# Autodesk Inventor assembly: Z-head-assembly-IKO-T1
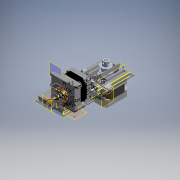
[picture p0: Inventor's stored thumbnail of the model, 180x180]
Saved by Autodesk Inventor 2016 (Build 200138000, 138)
## iProperties
Created: 2015-05-08
Part Number: Z-head-assembly-IKO-T1
Document SubType Name: Assembly
Designer: ax
Mass: 168.819 g
Surface Area: 717.643 cm^2
Volume: 138.854 cm^3
Density: 1.2158 g/cm^3
Author: ax
## Documents named in this file (24)
- C:\Users\as\Documents\Inventor\mintplacer-export\Z-head-assembly-IKO-T1.iam
- C:\Users\as\Documents\Inventor\mintplacer-export\Z-head-baseplate-IKO.ipt
- C:\Users\as\Documents\Inventor\mintplacer-export\BSPG15_60__40_.iam
- C:\Users\as\Documents\Inventor\mintplacer-export\C-head-base.ipt
- C:\Users\as\Documents\Inventor\mintplacer-export\C-head-side.ipt
- C:\Users\as\Documents\Inventor\mintplacer-export\GT2_20tooth.ipt
- C:\Users\as\Documents\Inventor\mintplacer-export\GT2-belt-2MR-200-06.ipt
- C:\Users\as\Documents\Inventor\mintplacer-export\HTD-5M-belt-clamp.ipt
- C:\Users\as\Documents\Inventor\mintplacer-export\GT2 belt clamp.ipt
- C:\Users\as\Documents\Inventor\mintplacer-export\NEMA14-Nanotec-ST3518S0804.ipt
- C:\Users\as\Documents\Inventor\mintplacer-export\nozzle-assembly.iam
- C:\Users\as\Documents\Inventor\mintplacer-export\Nanotec-ST4118S1404.iam
- C:\Users\as\Documents\Inventor\mintplacer-export\c-head-flange.ipt
- C:\Users\as\Documents\Inventor\mintplacer-export\Z-head-assembly-IKO-T1\Design Accelerator\Bolted Connection3.iam
- C:\Users\as\Documents\Inventor\mintplacer-export\Z-head-assembly-IKO-T1\Design Accelerator\Bolted Connection4.iam
- C:\Users\as\Documents\Inventor\mintplacer-export\Z-head-assembly-IKO-T1\Design Accelerator\Bolted Connection5.iam
- C:\Users\as\Documents\Inventor\mintplacer-export\Z-head-assembly-IKO-T1\Design Accelerator\Bolted Connection6.iam
- C:\Users\as\Documents\Inventor\mintplacer-export\Z-head-assembly-IKO-T1\Design Accelerator\Bolted Connection7.iam
- C:\Users\as\Documents\Inventor\mintplacer-export\small-tact-switch.ipt
- C:\Users\as\Documents\Inventor\mintplacer-export\Z-head-assembly-IKO-T1\Design Accelerator\Bolted Connection8.iam
- C:\Users\as\Documents\Inventor\mintplacer-export\Z-head-assembly-IKO-T1\Design Accelerator\Bolted Connection9.iam
- C:\Users\as\Documents\Inventor\mintplacer-export\Z-head-assembly-IKO-T1\Design Accelerator\Bolted Connection10.iam
- C:\Users\as\Documents\Inventor\mintplacer-export\Z-head-assembly-IKO-T1\Design Accelerator\Bolted Connection11.iam
- C:\Users\as\Documents\Inventor\Content Center Files\R2016\en-US\ISO 4762(1)\DIN EN ISO 4762 - M3 x 12.ipt
## Components (35 placed, 15 different names)
1. Z-head-baseplate-IKO:1 — Mate:1, Flush:1, Flush:2, Flush:7, Mate:5, Flush:9, Flush:10, Mate:10, Mate:37, Mate:38, Mate:39, Mate:40, Mate:41, Flush:21, Mate:70, Mate:71, Mate:74, Mate:76
2. HTD-5M-belt-clamp:1 — Flush:9, Flush:10
3. Nanotec-ST4118S1404:2 [sub-assembly] — Mate:5, Mate:10, Cylindrical:1, Flush:21, Mate:72, Mate:73, Mate:75
4. GT2_20tooth:1 — Mate:4, Cylindrical:1
5. BSPG15_60__40_:1 [sub-assembly] — Mate:1, Flush:1, Flush:2, Flush:3, Mate:11, Flush:19, Flush:20, Mate:43, Mate:69
6. c-head-flange:1 — Flush:14, Flush:15, Mate:11, Mate:12, Flush:17, Flush:19, Mate:32, Mate:33, Mate:34, Flush:20, Mate:42, Mate:47, Mate:52, Mate:53, Mate:68
7. C-head-base:1 — Flush:3, Flush:13, Mate:8, Mate:9, Flush:14, Flush:15, Flush:18, Mate:17, Mate:45
8. C-head-side:1 — Mate:7, Flush:11, Flush:13, Mate:12, Flush:17, Flush:18, Mate:17, Mate:44, Mate:46
9. NEMA14-Nanotec-ST3518S0804:1 — Mate:8, Mate:9
10. nozzle-assembly:1 [sub-assembly]
11. GT2 belt clamp:1 — Mate:7, Flush:11, Mate:48, Mate:49
12. Bolted Connection:3 [sub-assembly] — Mate:44, Mate:45
13. Bolted Connection:4 [sub-assembly] — Mate:46, Mate:47
14. Bolted Connection:5 [sub-assembly] — Mate:48, Mate:49
15. Bolted Connection:6 [sub-assembly] — Mate:68, Mate:69
16. Bolted Connection:7 [sub-assembly] — Mate:42, Mate:43
17. small-tact-switch:1 — Mate:32, Mate:33, Mate:34, Mate:62, Mate:63
18. Bolted Connection:8 [sub-assembly] — Mate:52, Mate:53
19. small-tact-switch:2 — Mate:37, Mate:38, Mate:66, Mate:67
20. small-tact-switch:3 — Mate:39, Mate:40, Mate:41, Mate:64, Mate:65
21. Bolted Connection:9 [sub-assembly] — Mate:62, Mate:63
22. Bolted Connection:10 [sub-assembly] — Mate:64, Mate:65
23. Bolted Connection:12 [sub-assembly] — Mate:66, Mate:67
24. DIN EN ISO 4762 M3 x 12:1 — Mate:70
25. DIN EN ISO 4762 M3 x 12:2 — Mate:71, Mate:72
26. DIN EN ISO 4762 M3 x 12:3 — Mate:74, Mate:75
27. DIN EN ISO 4762 M3 x 12:4 — Mate:73, Mate:76
28. GT2-belt-2MR-200-06:1 — Mate:4, Mate:6
29. GT2-belt-2MR-200-06:2
30. GT2-belt-2MR-200-06:3
31. GT2-belt-2MR-200-06:4
32. GT2-belt-2MR-200-06:5
33. GT2-belt-2MR-200-06:6
34. GT2-belt-2MR-200-06:7
35. GT2-belt-2MR-200-06:8
## Component patterns: (8 elements, first: GT2-belt-2MR-200-06:1)
## Relationships (61: Mate 44, Flush 16, CylindricalJoint 1)
- Mate:1: Z-head-baseplate-IKO:1 ↔ BSPG15_60__40_:1
- Flush:1: Z-head-baseplate-IKO:1 ↔ BSPG15_60__40_:1
- Flush:2: Z-head-baseplate-IKO:1 ↔ BSPG15_60__40_:1
- Flush:3: BSPG15_60__40_:1 ↔ C-head-base:1
- Mate:4 (1.4 mm): GT2_20tooth:1 ↔ GT2-belt-2MR-200-06:1
- Flush:7 (-6.3662 mm): Z-head-baseplate-IKO:1
- Mate:5 (-21 mm): Z-head-baseplate-IKO:1 ↔ Nanotec-ST4118S1404:2
- Flush:8 (-1.15 mm)
- Mate:6: GT2-belt-2MR-200-06:1
- Flush:9: Z-head-baseplate-IKO:1 ↔ HTD-5M-belt-clamp:1
- Flush:10: Z-head-baseplate-IKO:1 ↔ HTD-5M-belt-clamp:1
- Mate:7: C-head-side:1 ↔ GT2 belt clamp:1
- Flush:11: C-head-side:1 ↔ GT2 belt clamp:1
- Flush:13: C-head-base:1 ↔ C-head-side:1
- Mate:8: C-head-base:1 ↔ NEMA14-Nanotec-ST3518S0804:1
- Mate:9: C-head-base:1 ↔ NEMA14-Nanotec-ST3518S0804:1
- Mate:10: Z-head-baseplate-IKO:1 ↔ Nanotec-ST4118S1404:2
- Cylindrical:1: Nanotec-ST4118S1404:2 ↔ GT2_20tooth:1
- Flush:14: c-head-flange:1 ↔ C-head-base:1
- Flush:15: c-head-flange:1 ↔ C-head-base:1
- Mate:11: BSPG15_60__40_:1 ↔ c-head-flange:1
- Mate:12: c-head-flange:1 ↔ C-head-side:1
- Flush:17: c-head-flange:1 ↔ C-head-side:1
- Flush:18: C-head-base:1 ↔ C-head-side:1
- Flush:19: BSPG15_60__40_:1 ↔ c-head-flange:1
- Mate:17: C-head-base:1 ↔ C-head-side:1
- Mate:32: c-head-flange:1 ↔ small-tact-switch:1
- Mate:33: c-head-flange:1 ↔ small-tact-switch:1
- Mate:34: c-head-flange:1 ↔ small-tact-switch:1
- Flush:20: BSPG15_60__40_:1 ↔ c-head-flange:1
- Mate:37: Z-head-baseplate-IKO:1 ↔ small-tact-switch:2
- Mate:38: Z-head-baseplate-IKO:1 ↔ small-tact-switch:2
- Mate:39: Z-head-baseplate-IKO:1 ↔ small-tact-switch:3
- Mate:40: Z-head-baseplate-IKO:1 ↔ small-tact-switch:3
- Mate:41: Z-head-baseplate-IKO:1 ↔ small-tact-switch:3
- Mate:42: c-head-flange:1 ↔ Bolted Connection:7
- Mate:43: BSPG15_60__40_:1 ↔ Bolted Connection:7
- Mate:44: C-head-side:1 ↔ Bolted Connection:3
- Mate:45: C-head-base:1 ↔ Bolted Connection:3
- Mate:46: C-head-side:1 ↔ Bolted Connection:4
- Mate:47: c-head-flange:1 ↔ Bolted Connection:4
- Mate:48: GT2 belt clamp:1 ↔ Bolted Connection:5
- Mate:49: GT2 belt clamp:1 ↔ Bolted Connection:5
- Mate:52: c-head-flange:1 ↔ Bolted Connection:8
- Mate:53: c-head-flange:1 ↔ Bolted Connection:8
- Mate:62: small-tact-switch:1 ↔ Bolted Connection:9
- Mate:63: small-tact-switch:1 ↔ Bolted Connection:9
- Mate:64: small-tact-switch:3 ↔ Bolted Connection:10
- Mate:65: small-tact-switch:3 ↔ Bolted Connection:10
- Mate:66: small-tact-switch:2 ↔ Bolted Connection:12
- Mate:67: small-tact-switch:2 ↔ Bolted Connection:12
- Mate:68: c-head-flange:1 ↔ Bolted Connection:6
- Mate:69: BSPG15_60__40_:1 ↔ Bolted Connection:6
- Flush:21: Z-head-baseplate-IKO:1 ↔ Nanotec-ST4118S1404:2
- Mate:70: Z-head-baseplate-IKO:1 ↔ DIN EN ISO 4762 M3 x 12:1
- Mate:71: Z-head-baseplate-IKO:1 ↔ DIN EN ISO 4762 M3 x 12:2
- Mate:72: Nanotec-ST4118S1404:2 ↔ DIN EN ISO 4762 M3 x 12:2
- Mate:73: Nanotec-ST4118S1404:2 ↔ DIN EN ISO 4762 M3 x 12:4
- Mate:74: Z-head-baseplate-IKO:1 ↔ DIN EN ISO 4762 M3 x 12:3
- Mate:75: Nanotec-ST4118S1404:2 ↔ DIN EN ISO 4762 M3 x 12:3
- Mate:76: Z-head-baseplate-IKO:1 ↔ DIN EN ISO 4762 M3 x 12:4
## Named parameters: pulleyTeeth = 20, cPulley = 40 mm, dPulley = 12.7324 mm, beltThickness = 1.15 mm
